# Autodesk Inventor assembly: Servo Assembly
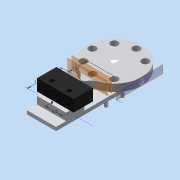
[picture p0: Inventor's stored thumbnail of the model, 180x180]
Saved by Autodesk Inventor 2017 SP1 (Build 210196100, 196)
## iProperties
Created: 2018-12-30
Part Number: Servo Assembly
Document SubType Name: Assembly
Designer: Dylan Rice
Author: Dylan Rice
## Documents named in this file (7)
- C:\Users\Dylan Rice\Documents\Current Projects\Project Sapo\Servo Things\Servo Mech CAD\Servo Assembly.iam
- C:\Users\Dylan Rice\Documents\Current Projects\Project Sapo\Servo Things\Servo Mech CAD\Encoder Front Plate.ipt
- C:\Users\Dylan Rice\Documents\Current Projects\Project Sapo\Servo Things\Servo Mech CAD\Housing front plate.ipt
- C:\Users\Dylan Rice\Documents\Current Projects\Project Sapo\Servo Things\Servo Mech CAD\Encoder Shaft.ipt
- C:\Users\Dylan Rice\Documents\Current Projects\Project Sapo\Servo Things\Servo Mech CAD\servo horn.ipt
- C:\Users\Dylan Rice\Documents\Current Projects\Project Sapo\Servo Things\Servo Mech CAD\Limit Switch.ipt
- C:\Users\Dylan Rice\Documents\Current Projects\Project Sapo\Servo Things\Servo Mech CAD\M1.6x0.35 Bolt.ipt
## Components (8 placed, 6 different names)
1. Encoder Front Plate:1 — Mate:13, Mate:14, Mate:15, Flush:3, Mate:16, Mate:17, Mate:18, Flush:4
2. Housing front plate:1 — Mate:10, Mate:11, Mate:12, Angle:1, Mate:13, Mate:14, Mate:15, Mate:19, Mate:21, Mate:22, Mate:23, Angle:2
3. Encoder Shaft:1 — Angle:1, Mate:18, Flush:4, Mate:24, Flush:5, Mate:25
4. servo horn:1 — Mate:24, Flush:5, Mate:25, Angle:2, Mate:26, Mate:27
5. Limit Switch:1 — Mate:10, Mate:11, Mate:12
6. M1.6x0.35 Bolt:1 — Mate:19, Mate:21
7. M1.6x0.35 Bolt:2 — Mate:22, Mate:23
8. M1.6x0.35 Bolt:3 — Mate:26, Mate:27
## Relationships (22: Mate 17, Flush 3, Angle 2)
- Mate:10: Housing front plate:1 ↔ Limit Switch:1
- Mate:11: Housing front plate:1 ↔ Limit Switch:1
- Mate:12: Housing front plate:1 ↔ Limit Switch:1
- Angle:1 (90 deg): Housing front plate:1 ↔ Encoder Shaft:1
- Mate:13: Encoder Front Plate:1 ↔ Housing front plate:1
- Mate:14: Encoder Front Plate:1 ↔ Housing front plate:1
- Mate:15: Encoder Front Plate:1 ↔ Housing front plate:1
- Flush:3: Encoder Front Plate:1
- Mate:16: Encoder Front Plate:1
- Mate:17: Encoder Front Plate:1
- Mate:18: Encoder Front Plate:1 ↔ Encoder Shaft:1
- Flush:4: Encoder Front Plate:1 ↔ Encoder Shaft:1
- Mate:19: Housing front plate:1 ↔ M1.6x0.35 Bolt:1
- Mate:21: Housing front plate:1 ↔ M1.6x0.35 Bolt:1
- Mate:22: Housing front plate:1 ↔ M1.6x0.35 Bolt:2
- Mate:23: Housing front plate:1 ↔ M1.6x0.35 Bolt:2
- Mate:24: Encoder Shaft:1 ↔ servo horn:1
- Flush:5: Encoder Shaft:1 ↔ servo horn:1
- Mate:25: Encoder Shaft:1 ↔ servo horn:1
- Angle:2 (180 deg): Housing front plate:1 ↔ servo horn:1
- Mate:26: servo horn:1 ↔ M1.6x0.35 Bolt:3
- Mate:27: servo horn:1 ↔ M1.6x0.35 Bolt:3
